# Autodesk Inventor assembly: Infrared sensor
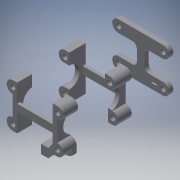
[picture p0: Inventor's stored thumbnail of the model, 180x180]
Saved by Autodesk Inventor 2019 (Build 230136000, 136)
## iProperties
Created: 2021-07-19
Part Number: Infrared sensor
Material: Типовые
Document SubType Name: Assembly
Designer: koryb
Author: koryb
## Documents named in this file (4)
- D:\AliasTrip\Inno Flying Platform 2021\Посадочная платформа\Зарядная Система\Тест\Infrared sensor.iam
- D:\AliasTrip\Inno Flying Platform 2021\Посадочная платформа\Зарядная Система\Тест\Base.ipt
- D:\AliasTrip\Inno Flying Platform 2021\Посадочная платформа\Зарядная Система\Тест\Fastening.ipt
- D:\AliasTrip\Inno Flying Platform 2021\Посадочная платформа\Зарядная Система\Тест\Fastening back.ipt
## Components (3 placed, 3 different names)
1. Base:1 — Заподлицо:1
2. Fastening:1 — Заподлицо:1, Совмещение:1, Заподлицо:2, Заподлицо:3
3. Fastening back:1 — Совмещение:1, Заподлицо:2, Заподлицо:3
## Relationships (4: Flush 3, Mate 1)
- Заподлицо:1 [Flush] (25 mm): Base:1 ↔ Fastening:1
- Совмещение:1 [Mate] (25 mm): Fastening:1 ↔ Fastening back:1
- Заподлицо:2 [Flush]: Fastening:1 ↔ Fastening back:1
- Заподлицо:3 [Flush]: Fastening:1 ↔ Fastening back:1
